# Autodesk Inventor assembly: Cathode Flange
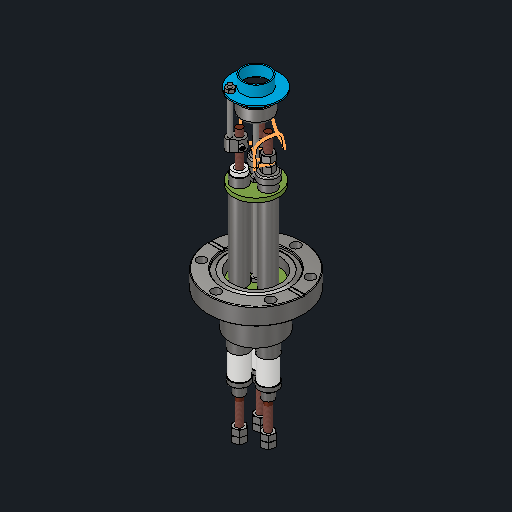
[picture p0: Inventor's stored thumbnail of the model, 512x512]
Saved by Autodesk Inventor 2026 (Build 300175050, 175E)
## iProperties
Created: 2024-05-14
Part Number: Cathode Flange
Document SubType Name: Assembly
Designer: KAA
Author: KAA
## Documents named in this file (16)
- C:\Users\queez\Dropbox\Drawings\PIHTI\Plasma Vessel\Cathode-Anode-Flange\Cathode-Anode-70IC-flange-with-feeds.iam
- C:\Users\queez\Dropbox\Drawings\PIHTI\Plasma Vessel\Cathode-Anode-Flange\cf70_three-feed_flange.ipt
- C:\Users\queez\Dropbox\Drawings\PIHTI\Plasma Vessel\Cathode-Anode-Flange\copper-feed\HighCurrentFeed.iam
- C:\Users\queez\Dropbox\Drawings\PIHTI\ContentCenter\Fastners\m5-nut.ipt
- C:\Users\queez\Dropbox\Drawings\PIHTI\ContentCenter\Ceramics\Ceramic-Cylinder-10x6x10.ipt
- C:\Users\queez\Dropbox\Drawings\PIHTI\Plasma Vessel\Cathode-Anode-Flange\ring-pre-anode.ipt
- C:\Users\queez\Dropbox\Drawings\PIHTI\Plasma Vessel\Cathode-Anode-Flange\cathode-screen-v0.ipt
- C:\Users\queez\Dropbox\Drawings\PIHTI\Plasma Vessel\Cathode-Anode-Flange\electrode-skirt-pipe.ipt
- C:\Users\queez\Dropbox\Drawings\PIHTI\Plasma Vessel\Cathode-Anode-Flange\electrode-aligning-disk.ipt
- C:\Users\queez\Dropbox\Drawings\PIHTI\Plasma Vessel\Cathode-Anode-Flange\m3-pin-for-ring-anode.ipt
- C:\Users\queez\Dropbox\Drawings\PIHTI\ContentCenter\Fastners\M3-nut.ipt
- C:\Users\queez\Dropbox\Drawings\PIHTI\Plasma Vessel\Cathode-Anode-Flange\m3-pin-for-cathode-skirt.ipt
- C:\Users\queez\Dropbox\Drawings\PIHTI\Plasma Vessel\Cathode-Anode-Flange\anode-holding-nut.ipt
- C:\Users\queez\Dropbox\Drawings\PIHTI\ContentCenter\Fastners\M3x5-set-screw.ipt
- C:\Users\queez\Dropbox\Drawings\PIHTI\Plasma Vessel\Cathode-Anode-Flange\electrode-skirt-short.ipt
- C:\Users\queez\Dropbox\Drawings\PIHTI\Plasma Vessel\Cathode-Anode-Flange\Cathode-tungsten-wire-v3-filament-solid.ipt
## Components (70 placed, 15 different names)
1. cf70_three-feed_flange:1 — Flush:1, Mate:1, Flush:2, Rigid:1, Rigid:2, Rigid:3, Mate:12, Mate:13, Mate:30, Mate:38, Mate:40
2. HighCurrentFeed:1 [sub-assembly] — Rigid:1, Rotational:4, Rigid:4, Mate:33, Mate:35, Mate:48
3. HighCurrentFeed:2 [sub-assembly] — Rigid:2, Rotational:5, Mate:5, Mate:6, Rotational:9, Mate:34, Mate:37, Mate:52
4. HighCurrentFeed:3 [sub-assembly] — Rigid:3, Rotational:3, Mate:3, Mate:4, Rigid:5, Mate:32, Mate:36, Mate:39, Mate:41, Mate:53
5. ring-pre-anode:1 — Mate:12, Mate:13, Mate:19, Mate:42, Rigid:31, Rigid:32
6. cathode-screen-v0:1 — Mate:30, Rotational:13, Rotational:15
7. electrode-skirt-pipe:1 — Mate:32, Mate:36
8. electrode-skirt-pipe:2 — Mate:33, Mate:35
9. electrode-skirt-pipe:3 — Mate:34, Mate:37
10. electrode-aligning-disk:1 — Mate:38, Mate:39, Rotational:14, Rigid:33
11. electrode-aligning-disk:2 — Mate:40, Mate:41, Mate:43, Mate:45, Mate:47
12. m3-pin-for-ring-anode:1 — Mate:42, Flush:6, Mate:49
13. m3-pin-for-cathode-skirt:1 — Mate:43, Mate:44, Mate:46
14. anode-holding-nut:1 — Mate:48, Mate:49, Mate:50, Mate:51, Rigid:37, Rigid:38
15. Ceramic-Cylinder-10x6x10:31 — Rigid:34, Rotational:16
16. Ceramic-Cylinder-10x6x10:32 — Rigid:35, Rotational:18
17. Ceramic-Cylinder-10x6x10:33 — Rigid:36
18. electrode-skirt-short:2 — Rotational:18
19. electrode-skirt-short:3 — Rotational:16
20. Cathode-tungsten-wire-v3-filament-solid:1 — Mate:52, Mate:53
21. Ceramic-Cylinder-10x6x10:26 — Rotational:12, Rigid:28
22. Ceramic-Cylinder-10x6x10:27 — Rigid:27, Rigid:30
23. Ceramic-Cylinder-10x6x10:28 — Rigid:28, Rigid:35
24. Ceramic-Cylinder-10x6x10:29 — Rigid:29, Rigid:36
25. Ceramic-Cylinder-10x6x10:30 — Rigid:30, Rigid:34
26. Ceramic-Cylinder-10x6x10:1 — Rigid:4, Rigid:7
27. Ceramic-Cylinder-10x6x10:2 — Rigid:8, Rigid:9
28. Ceramic-Cylinder-10x6x10:3 — Rigid:7, Rigid:10
29. Ceramic-Cylinder-10x6x10:4 — Rotational:9, Rigid:6
30. Ceramic-Cylinder-10x6x10:5 — Rigid:6, Rigid:8
31. Ceramic-Cylinder-10x6x10:6 — Rigid:5, Rigid:26
32. Ceramic-Cylinder-10x6x10:7 — Rigid:15, Rigid:17
33. Ceramic-Cylinder-10x6x10:8 — Rigid:12, Rigid:16
34. Ceramic-Cylinder-10x6x10:9 — Rigid:10, Rigid:12
35. Ceramic-Cylinder-10x6x10:10 — Rigid:26, Rigid:11
36. Ceramic-Cylinder-10x6x10:11 — Rigid:16, Rotational:11
37. Ceramic-Cylinder-10x6x10:12 — Rigid:17, Rigid:19
38. Ceramic-Cylinder-10x6x10:13 — Rigid:18, Rigid:21
39. Ceramic-Cylinder-10x6x10:14 — Rigid:14, Rigid:18
40. Ceramic-Cylinder-10x6x10:15 — Rigid:13, Rigid:15
41. Ceramic-Cylinder-10x6x10:16 — Rigid:11, Rigid:13
42. Ceramic-Cylinder-10x6x10:17 — Rigid:9, Rigid:14
43. Ceramic-Cylinder-10x6x10:18 — Rotational:11, Rigid:20
44. Ceramic-Cylinder-10x6x10:19 — Rigid:19, Rigid:22
45. Ceramic-Cylinder-10x6x10:20 — Rigid:21, Rigid:24
46. Ceramic-Cylinder-10x6x10:21 — Rigid:25, Rigid:29
47. Ceramic-Cylinder-10x6x10:22 — Rigid:23, Rigid:25
48. Ceramic-Cylinder-10x6x10:23 — Rigid:24, Rotational:12
49. Ceramic-Cylinder-10x6x10:24 — Rigid:20, Rigid:23
50. Ceramic-Cylinder-10x6x10:25 — Rigid:22, Rigid:27
51. JIS B 1181 Style 1 - Metric A M3:8 — Rotational:15
52. CNS 4480 M3 x 5:1 — Mate:50, Rigid:38
53. CNS 4480 M3 x 5:2 — Mate:51, Rigid:37
54. JIS B 1181 Style 1 - Metric A M3:4 — Mate:46, Mate:47
55. JIS B 1181 Style 1 - Metric A M3:5 — Rotational:13
56. JIS B 1181 Style 1 - Metric A M3:6 — Rotational:14
57. JIS B 1181 Style 1 - Metric A M3:7 — Rigid:33
58. JIS B 1181 Style 1 - Metric A M3:1 — Rigid:31, Flush:6
59. JIS B 1181 Style 1 - Metric A M3:2 — Rigid:32
60. JIS B 1181 Style 1 - Metric A M3:3 — Mate:44, Mate:45
61. Hex Nut Metric M5 x 0,8:3 — Mate:3
62. Hex Nut Metric M5 x 0,8:4 — Mate:4
63. Hex Nut Metric M5 x 0,8:5 — Mate:5
64. Hex Nut Metric M5 x 0,8:6 — Mate:6
65. Hex Nut Metric M5 x 0,8:7 — Rotational:4, Rotational:7
66. Hex Nut Metric M5 x 0,8:8 — Rotational:8
67. Hex Nut Metric M5 x 0,8:9 — Rotational:6
68. Hex Nut Metric M5 x 0,8:10 — Rotational:5, Rotational:8
69. Hex Nut Metric M5 x 0,8:11 — Rotational:3, Rotational:6
70. Hex Nut Metric M5 x 0,8:12 — Rotational:7
## Relationships (86: WeldJoint 38, Mate 31, RevoluteJoint 14, Flush 3)
- Flush:1: cf70_three-feed_flange:1
- Mate:1: cf70_three-feed_flange:1
- Flush:2: cf70_three-feed_flange:1
- Rigid:1 [WeldJoint]: cf70_three-feed_flange:1 ↔ HighCurrentFeed:1
- Rigid:2 [WeldJoint]: cf70_three-feed_flange:1 ↔ HighCurrentFeed:2
- Rigid:3 [WeldJoint]: cf70_three-feed_flange:1 ↔ HighCurrentFeed:3
- Rotational:3 [RevoluteJoint]: HighCurrentFeed:3 ↔ Hex Nut Metric M5 x 0,8:11
- Rotational:4 [RevoluteJoint]: HighCurrentFeed:1 ↔ Hex Nut Metric M5 x 0,8:7
- Rotational:5 [RevoluteJoint]: HighCurrentFeed:2 ↔ Hex Nut Metric M5 x 0,8:10
- Rotational:6 [RevoluteJoint]: Hex Nut Metric M5 x 0,8:9 ↔ Hex Nut Metric M5 x 0,8:11
- Rotational:7 [RevoluteJoint]: Hex Nut Metric M5 x 0,8:7 ↔ Hex Nut Metric M5 x 0,8:12
- Rotational:8 [RevoluteJoint]: Hex Nut Metric M5 x 0,8:8 ↔ Hex Nut Metric M5 x 0,8:10
- Mate:3: HighCurrentFeed:3 ↔ Hex Nut Metric M5 x 0,8:3
- Mate:4: HighCurrentFeed:3 ↔ Hex Nut Metric M5 x 0,8:4
- Mate:5: HighCurrentFeed:2 ↔ Hex Nut Metric M5 x 0,8:5
- Mate:6: HighCurrentFeed:2 ↔ Hex Nut Metric M5 x 0,8:6
- Rigid:4 [WeldJoint]: HighCurrentFeed:1 ↔ Ceramic-Cylinder-10x6x10:1
- Rotational:9 [RevoluteJoint]: HighCurrentFeed:2 ↔ Ceramic-Cylinder-10x6x10:4
- Rigid:5 [WeldJoint]: HighCurrentFeed:3 ↔ Ceramic-Cylinder-10x6x10:6
- Rigid:6 [WeldJoint]: Ceramic-Cylinder-10x6x10:4 ↔ Ceramic-Cylinder-10x6x10:5
- Rigid:7 [WeldJoint]: Ceramic-Cylinder-10x6x10:1 ↔ Ceramic-Cylinder-10x6x10:3
- Rigid:8 [WeldJoint]: Ceramic-Cylinder-10x6x10:2 ↔ Ceramic-Cylinder-10x6x10:5
- Rigid:26 [WeldJoint]: Ceramic-Cylinder-10x6x10:6 ↔ Ceramic-Cylinder-10x6x10:10
- Rigid:9 [WeldJoint]: Ceramic-Cylinder-10x6x10:2 ↔ Ceramic-Cylinder-10x6x10:17
- Rigid:10 [WeldJoint]: Ceramic-Cylinder-10x6x10:3 ↔ Ceramic-Cylinder-10x6x10:9
- Rigid:11 [WeldJoint]: Ceramic-Cylinder-10x6x10:10 ↔ Ceramic-Cylinder-10x6x10:16
- Rigid:12 [WeldJoint]: Ceramic-Cylinder-10x6x10:8 ↔ Ceramic-Cylinder-10x6x10:9
- Rigid:13 [WeldJoint]: Ceramic-Cylinder-10x6x10:15 ↔ Ceramic-Cylinder-10x6x10:16
- Rigid:14 [WeldJoint]: Ceramic-Cylinder-10x6x10:14 ↔ Ceramic-Cylinder-10x6x10:17
- Rigid:15 [WeldJoint]: Ceramic-Cylinder-10x6x10:7 ↔ Ceramic-Cylinder-10x6x10:15
- Rigid:16 [WeldJoint]: Ceramic-Cylinder-10x6x10:8 ↔ Ceramic-Cylinder-10x6x10:11
- Rigid:17 [WeldJoint]: Ceramic-Cylinder-10x6x10:7 ↔ Ceramic-Cylinder-10x6x10:12
- Rigid:18 [WeldJoint]: Ceramic-Cylinder-10x6x10:13 ↔ Ceramic-Cylinder-10x6x10:14
- Rotational:11 [RevoluteJoint]: Ceramic-Cylinder-10x6x10:11 ↔ Ceramic-Cylinder-10x6x10:18
- Rigid:19 [WeldJoint]: Ceramic-Cylinder-10x6x10:12 ↔ Ceramic-Cylinder-10x6x10:19
- Rigid:20 [WeldJoint]: Ceramic-Cylinder-10x6x10:18 ↔ Ceramic-Cylinder-10x6x10:24
- Rigid:21 [WeldJoint]: Ceramic-Cylinder-10x6x10:13 ↔ Ceramic-Cylinder-10x6x10:20
- Rigid:22 [WeldJoint]: Ceramic-Cylinder-10x6x10:19 ↔ Ceramic-Cylinder-10x6x10:25
- Rigid:23 [WeldJoint]: Ceramic-Cylinder-10x6x10:22 ↔ Ceramic-Cylinder-10x6x10:24
- Rigid:24 [WeldJoint]: Ceramic-Cylinder-10x6x10:20 ↔ Ceramic-Cylinder-10x6x10:23
- Rigid:25 [WeldJoint]: Ceramic-Cylinder-10x6x10:21 ↔ Ceramic-Cylinder-10x6x10:22
- Rotational:12 [RevoluteJoint]: Ceramic-Cylinder-10x6x10:26 ↔ Ceramic-Cylinder-10x6x10:23
- Rigid:27 [WeldJoint]: Ceramic-Cylinder-10x6x10:27 ↔ Ceramic-Cylinder-10x6x10:25
- Rigid:28 [WeldJoint]: Ceramic-Cylinder-10x6x10:26 ↔ Ceramic-Cylinder-10x6x10:28
- Rigid:29 [WeldJoint]: Ceramic-Cylinder-10x6x10:29 ↔ Ceramic-Cylinder-10x6x10:21
- Rigid:30 [WeldJoint]: Ceramic-Cylinder-10x6x10:27 ↔ Ceramic-Cylinder-10x6x10:30
- Mate:12: cf70_three-feed_flange:1 ↔ ring-pre-anode:1
- Mate:13 (115 mm): cf70_three-feed_flange:1 ↔ ring-pre-anode:1
- Mate:19: ring-pre-anode:1
- Mate:30: cf70_three-feed_flange:1 ↔ cathode-screen-v0:1
- Mate:32: HighCurrentFeed:3 ↔ electrode-skirt-pipe:1
- Mate:33: HighCurrentFeed:1 ↔ electrode-skirt-pipe:2
- Mate:34: HighCurrentFeed:2 ↔ electrode-skirt-pipe:3
- Mate:35: HighCurrentFeed:1 ↔ electrode-skirt-pipe:2
- Mate:36: HighCurrentFeed:3 ↔ electrode-skirt-pipe:1
- Mate:37: HighCurrentFeed:2 ↔ electrode-skirt-pipe:3
- Mate:38: cf70_three-feed_flange:1 ↔ electrode-aligning-disk:1
- Mate:39: HighCurrentFeed:3 ↔ electrode-aligning-disk:1
- Mate:40: cf70_three-feed_flange:1 ↔ electrode-aligning-disk:2
- Mate:41: HighCurrentFeed:3 ↔ electrode-aligning-disk:2
- Mate:42: ring-pre-anode:1 ↔ m3-pin-for-ring-anode:1
- Rigid:31 [WeldJoint]: ring-pre-anode:1 ↔ JIS B 1181 Style 1 - Metric A M3:1
- Rigid:32 [WeldJoint]: ring-pre-anode:1 ↔ JIS B 1181 Style 1 - Metric A M3:2
- Flush:6 (-2 mm): m3-pin-for-ring-anode:1 ↔ JIS B 1181 Style 1 - Metric A M3:1
- Mate:43: electrode-aligning-disk:2 ↔ m3-pin-for-cathode-skirt:1
- Mate:44: m3-pin-for-cathode-skirt:1 ↔ JIS B 1181 Style 1 - Metric A M3:3
- Mate:45: electrode-aligning-disk:2 ↔ JIS B 1181 Style 1 - Metric A M3:3
- Mate:46: m3-pin-for-cathode-skirt:1 ↔ JIS B 1181 Style 1 - Metric A M3:4
- Mate:47: electrode-aligning-disk:2 ↔ JIS B 1181 Style 1 - Metric A M3:4
- Rotational:13 [RevoluteJoint]: cathode-screen-v0:1 ↔ JIS B 1181 Style 1 - Metric A M3:5
- Rotational:14 [RevoluteJoint]: electrode-aligning-disk:1 ↔ JIS B 1181 Style 1 - Metric A M3:6
- Rigid:33 [WeldJoint]: electrode-aligning-disk:1 ↔ JIS B 1181 Style 1 - Metric A M3:7
- Mate:48: HighCurrentFeed:1 ↔ anode-holding-nut:1
- Mate:49: m3-pin-for-ring-anode:1 ↔ anode-holding-nut:1
- Rotational:15 [RevoluteJoint]: cathode-screen-v0:1 ↔ JIS B 1181 Style 1 - Metric A M3:8
- Rigid:34 [WeldJoint]: Ceramic-Cylinder-10x6x10:31 ↔ Ceramic-Cylinder-10x6x10:30
- Rigid:35 [WeldJoint]: Ceramic-Cylinder-10x6x10:32 ↔ Ceramic-Cylinder-10x6x10:28
- Rigid:36 [WeldJoint]: Ceramic-Cylinder-10x6x10:33 ↔ Ceramic-Cylinder-10x6x10:29
- Mate:50: anode-holding-nut:1 ↔ CNS 4480 M3 x 5:1
- Mate:51: anode-holding-nut:1 ↔ CNS 4480 M3 x 5:2
- Rigid:37 [WeldJoint]: anode-holding-nut:1 ↔ CNS 4480 M3 x 5:2
- Rigid:38 [WeldJoint]: anode-holding-nut:1 ↔ CNS 4480 M3 x 5:1
- Rotational:16 [RevoluteJoint]: Ceramic-Cylinder-10x6x10:31 ↔ electrode-skirt-short:3
- Rotational:18 [RevoluteJoint]: Ceramic-Cylinder-10x6x10:32 ↔ electrode-skirt-short:2
- Mate:52: HighCurrentFeed:2 ↔ Cathode-tungsten-wire-v3-filament-solid:1
- Mate:53: HighCurrentFeed:3 ↔ Cathode-tungsten-wire-v3-filament-solid:1
